# Autodesk Inventor assembly: Extrusor
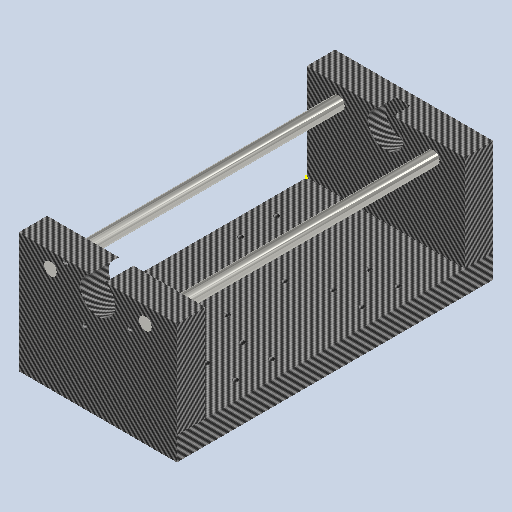
[picture p0: Inventor's stored thumbnail of the model, 512x512]
Saved by Autodesk Inventor 2022.2 (Build 262287000, 287)
## iProperties
Created: 2021-11-08
Part Number: Extrusor
Document SubType Name: Assembly
Designer: Samuel Gómez
Author: Samuel Gómez
## Documents named in this file (5)
- E:\Samuel Gómez\Documentos\ITM\Cuarto Semestre\Dibujo\Final\Original\Trabajo Final Impresora 3D\Extrusor.iam
- E:\Samuel Gómez\Documentos\ITM\Cuarto Semestre\Dibujo\Final\Original\Trabajo Final Impresora 3D\Placa6 Base1.ipt
- E:\Samuel Gómez\Documentos\ITM\Cuarto Semestre\Dibujo\Final\Original\Trabajo Final Impresora 3D\Placa6 Base3.ipt
- E:\Samuel Gómez\Documentos\ITM\Cuarto Semestre\Dibujo\Final\Original\Trabajo Final Impresora 3D\Placa6 Base2.ipt
- E:\Samuel Gómez\Documentos\ITM\Cuarto Semestre\Dibujo\Final\Original\Trabajo Final Impresora 3D\Varilla 200.ipt
## Components (5 placed, 4 different names)
1. Placa6 Base1:1 — Coincidencia:1, Nivelación:1, Nivelación:2
2. Placa6 Base3:1 — Coincidencia:1, Nivelación:1, Nivelación:2, Nivelación:3, Coincidencia:2, Nivelación:4
3. Placa6 Base2:1 — Nivelación:3, Coincidencia:2, Nivelación:4, Coincidencia:3, Coincidencia:4, Nivelación:5, Nivelación:6
4. Varilla 200:1 — Coincidencia:3, Nivelación:6
5. Varilla 200:2 — Coincidencia:4, Nivelación:5
## Relationships (10: Flush 6, Mate 4)
- Coincidencia:1 [Mate]: Placa6 Base1:1 ↔ Placa6 Base3:1
- Nivelación:1 [Flush]: Placa6 Base1:1 ↔ Placa6 Base3:1
- Nivelación:2 [Flush]: Placa6 Base1:1 ↔ Placa6 Base3:1
- Nivelación:3 [Flush]: Placa6 Base3:1 ↔ Placa6 Base2:1
- Coincidencia:2 [Mate]: Placa6 Base3:1 ↔ Placa6 Base2:1
- Nivelación:4 [Flush]: Placa6 Base3:1 ↔ Placa6 Base2:1
- Coincidencia:3 [Mate]: Placa6 Base2:1 ↔ Varilla 200:1
- Coincidencia:4 [Mate]: Placa6 Base2:1 ↔ Varilla 200:2
- Nivelación:5 [Flush]: Placa6 Base2:1 ↔ Varilla 200:2
- Nivelación:6 [Flush]: Placa6 Base2:1 ↔ Varilla 200:1
